# Autodesk Inventor assembly: Case assembled
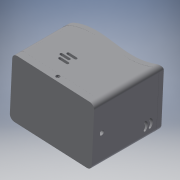
[picture p0: Inventor's stored thumbnail of the model, 180x180]
Saved by Autodesk Inventor 2019 (Build 230136000, 136)
## iProperties
Created: 2022-04-25
Part Number: Case assembled
Document SubType Name: Assembly
Designer: Loxei
Author: Loxei
## Documents named in this file (7)
- C:\Users\Loxei\Documents\High School\Sophomore\-CNED-\Engineering\Work\6\3D\Case assembled.iam
- C:\Users\Loxei\Documents\High School\Sophomore\-CNED-\Engineering\Work\6\3D\Case Back.ipt
- C:\Users\Loxei\Documents\High School\Sophomore\-CNED-\Engineering\Work\6\3D\Case Bottom.ipt
- C:\Users\Loxei\Documents\High School\Sophomore\-CNED-\Engineering\Work\6\3D\Case Front.ipt
- C:\Users\Loxei\Documents\High School\Sophomore\-CNED-\Engineering\Work\6\3D\Case Left.ipt
- C:\Users\Loxei\Documents\High School\Sophomore\-CNED-\Engineering\Work\6\3D\Case Right.ipt
- C:\Users\Loxei\Documents\High School\Sophomore\-CNED-\Engineering\Work\6\3D\Case Top.ipt
## Components (6 placed, 6 different names)
1. Case Bottom:1 — Rigid:1, Mate:3, Mate:7, Mate:8
2. Case Back:1 — Mate:2, Mate:3, Mate:9
3. Case Front:1 — Rigid:1, Mate:4, Mate:5, Mate:6
4. Case Left:1 — Mate:2, Mate:6, Mate:7
5. Case Right:1 — Mate:8, Mate:9
6. Case Top:1 — Mate:4, Mate:5
## Relationships (9: Mate 8, WeldJoint 1)
- Rigid:1 [WeldJoint]: Case Bottom:1 ↔ Case Front:1
- Mate:2: Case Back:1 ↔ Case Left:1
- Mate:3: Case Bottom:1 ↔ Case Back:1
- Mate:4: Case Front:1 ↔ Case Top:1
- Mate:5: Case Front:1 ↔ Case Top:1
- Mate:6: Case Front:1 ↔ Case Left:1
- Mate:7: Case Bottom:1 ↔ Case Left:1
- Mate:8: Case Bottom:1 ↔ Case Right:1
- Mate:9: Case Back:1 ↔ Case Right:1
